# Autodesk Inventor assembly: Сборка_Концепт
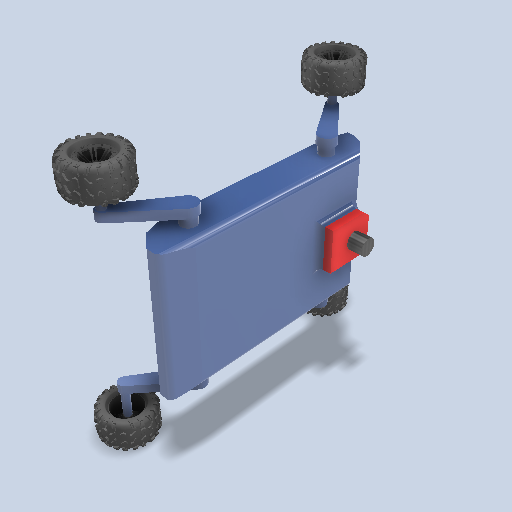
[picture p0: Inventor's stored thumbnail of the model, 512x512]
Saved by Autodesk Inventor 2025 (Build 290162000, 162)
## iProperties
Created: 2025-12-16
Part Number: Сборка_Концепт
Document SubType Name: Assembly
Designer: Artem Sannikov
Author: Artem Sannikov
## Documents named in this file (4)
- C:\Users\Artem Sannikov\Desktop\Robo-Forester\3D\Сборка_Концепт.iam
- C:\Users\Artem Sannikov\Desktop\Robo-Forester\3D\car_wheel2.ipt
- C:\Users\Artem Sannikov\Desktop\Robo-Forester\3D\Body.ipt
- C:\Users\Artem Sannikov\Desktop\Robo-Forester\3D\car_wheel2_MIR.ipt
## Components (5 placed, 3 different names)
1. car_wheel2:1 — Заподлицо:1
2. Body:1 — Заподлицо:1, Совмещение:1, Совмещение:2
3. car_wheel2:2 — Совмещение:1, Совмещение:2
4. car_wheel2_MIR:1
5. car_wheel2_MIR:2
## Relationships (3: Mate 2, Flush 1)
- Заподлицо:1 [Flush]: car_wheel2:1 ↔ Body:1
- Совмещение:1 [Mate]: Body:1 ↔ car_wheel2:2
- Совмещение:2 [Mate]: Body:1 ↔ car_wheel2:2
